# Autodesk Inventor assembly: EnsembleAvant
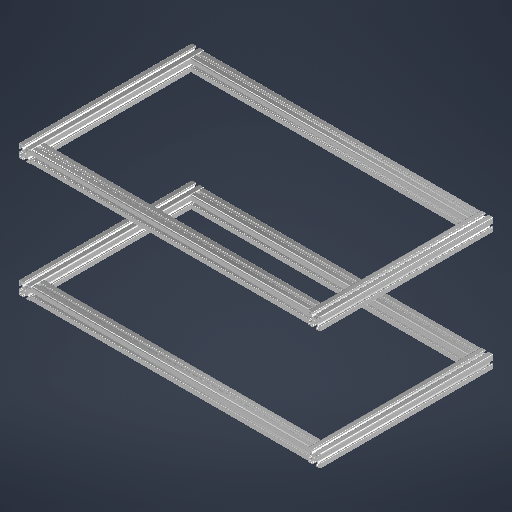
[picture p0: Inventor's stored thumbnail of the model, 512x512]
Saved by Autodesk Inventor 2026.2 (Build 302298010, 298A)
## iProperties
Part Number: EnsembleAvant
Document SubType Name: Ensemble
Designer: quent
Author: quent
## Documents named in this file (3)
- C:\Users\quent\OneDrive\Bureau\Master 2\Q2\Projet\EcoShell3D_VF\EnsembleAvant.iam
- C:\Users\quent\OneDrive\Bureau\Master 2\Q2\Projet\EcoShell3D_VF\profileAluAvant2.ipt
- C:\Users\quent\OneDrive\Bureau\Master 2\Q2\Projet\EcoShell3D_VF\profileAluAvant1.ipt
## Components (8 placed, 2 different names)
1. profileAluAvant2:1 — Placage:1, Affleurement:1, Affleurement:2, Affleurement:3, Affleurement:5, Placage:3, Affleurement:6, Affleurement:7, Placage:4, Placage:6
2. profileAluAvant2:2 — Placage:1, Affleurement:1, Affleurement:2, Affleurement:3, Placage:2, Affleurement:4, Affleurement:8, Affleurement:13, Affleurement:14
3. profileAluAvant2:3 — Placage:2, Affleurement:4, Affleurement:9, Affleurement:10, Placage:5, Affleurement:15, Affleurement:16, Placage:7
4. profileAluAvant2:4 — Affleurement:5, Placage:3, Affleurement:11
5. profileAluAvant1:1 — Affleurement:9, Affleurement:10, Placage:5, Affleurement:11, Affleurement:12
6. profileAluAvant1:2 — Affleurement:6, Affleurement:7, Placage:4, Affleurement:8, Affleurement:12
7. profileAluAvant1:3 — Affleurement:15, Affleurement:16, Placage:7
8. profileAluAvant1:4 — Affleurement:13, Affleurement:14, Placage:6
## Relationships (23: Flush 16, Mate 7)
- Placage:1 [Mate] (632 mm): profileAluAvant2:1 ↔ profileAluAvant2:2
- Affleurement:1 [Flush]: profileAluAvant2:1 ↔ profileAluAvant2:2
- Affleurement:2 [Flush]: profileAluAvant2:1 ↔ profileAluAvant2:2
- Affleurement:3 [Flush]: profileAluAvant2:1 ↔ profileAluAvant2:2
- Placage:2 [Mate] (241.624 mm): profileAluAvant2:2 ↔ profileAluAvant2:3
- Affleurement:4 [Flush]: profileAluAvant2:2 ↔ profileAluAvant2:3
- Affleurement:5 [Flush]: profileAluAvant2:1 ↔ profileAluAvant2:4
- Placage:3 [Mate] (241.624 mm): profileAluAvant2:1 ↔ profileAluAvant2:4
- Affleurement:6 [Flush]: profileAluAvant2:1 ↔ profileAluAvant1:2
- Affleurement:7 [Flush]: profileAluAvant2:1 ↔ profileAluAvant1:2
- Placage:4 [Mate]: profileAluAvant2:1 ↔ profileAluAvant1:2
- Affleurement:8 [Flush]: profileAluAvant2:2 ↔ profileAluAvant1:2
- Affleurement:9 [Flush]: profileAluAvant2:3 ↔ profileAluAvant1:1
- Affleurement:10 [Flush]: profileAluAvant2:3 ↔ profileAluAvant1:1
- Placage:5 [Mate]: profileAluAvant2:3 ↔ profileAluAvant1:1
- Affleurement:11 [Flush]: profileAluAvant2:4 ↔ profileAluAvant1:1
- Affleurement:12 [Flush]: profileAluAvant1:1 ↔ profileAluAvant1:2
- Affleurement:13 [Flush]: profileAluAvant2:2 ↔ profileAluAvant1:4
- Affleurement:14 [Flush]: profileAluAvant2:2 ↔ profileAluAvant1:4
- Placage:6 [Mate]: profileAluAvant2:1 ↔ profileAluAvant1:4
- Affleurement:15 [Flush]: profileAluAvant2:3 ↔ profileAluAvant1:3
- Affleurement:16 [Flush]: profileAluAvant2:3 ↔ profileAluAvant1:3
- Placage:7 [Mate]: profileAluAvant2:3 ↔ profileAluAvant1:3
